# Autodesk Inventor assembly: 217-2428-200 Rev1
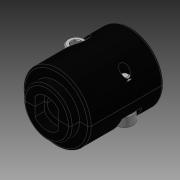
[picture p0: Inventor's stored thumbnail of the model, 180x180]
Saved by Autodesk Inventor 2014 SP1 (Build 180222100, 222)
## iProperties
Created: 2014-01-07
Part Number: 217-2428-200 Rev1
Document SubType Name: Assembly
Designer: Andrew Toennies
Mass: 35.4945 g
Surface Area: 37.4009 cm^2
Volume: 4.52159 cm^3
Density: 7.85 g/cm^3
Author: Andrew Toennies
## Documents named in this file (4)
- C:\Users\Moses\Documents\GitHub\2014buildCAD\Shooter\Constrained 2 Speed Ball Shifter\217-2428-200 Rev1.iam
- C:\Users\Moses\Documents\GitHub\2014buildCAD\Shooter\Constrained 2 Speed Ball Shifter\217-2428-032 Rev1.ipt
- C:\Users\Moses\Documents\GitHub\2014buildCAD\Shooter\Constrained 2 Speed Ball Shifter\217-2778-NCQ8A075-050M_1032_Nut_90545A111.ipt
- C:\Users\Moses\Documents\GitHub\2014buildCAD\Shooter\Constrained 2 Speed Ball Shifter\91251A107_91251A107.ipt
## Components (5 placed, 5 different names)
1. 217-2428-032 Rev1_50 — Insert:2, Mate:2, Mate:3
2. 217-2428-032 Rev1_51 — Insert:1, Mate:1, Angle:1, Mate:2, Mate:3
3. 217-2778-NCQ8A075-050M_1032_Nut_90545A111_52 — Mate:1, Angle:1
4. 91251A107_91251A107_53 — Insert:2
5. 91251A107_91251A107_54 — Insert:1
## Relationships (6: Mate 3, Insert 2, Angle 1)
- Insert:1: 217-2428-032 Rev1_51 ↔ 91251A107_91251A107_54
- Insert:2: 217-2428-032 Rev1_50 ↔ 91251A107_91251A107_53
- Mate:1: 217-2428-032 Rev1_51 ↔ 217-2778-NCQ8A075-050M_1032_Nut_90545A111_52
- Angle:1 (0 deg): 217-2428-032 Rev1_51 ↔ 217-2778-NCQ8A075-050M_1032_Nut_90545A111_52
- Mate:2: 217-2428-032 Rev1_50 ↔ 217-2428-032 Rev1_51
- Mate:3: 217-2428-032 Rev1_50 ↔ 217-2428-032 Rev1_51
